# Autodesk Inventor assembly: side_channel
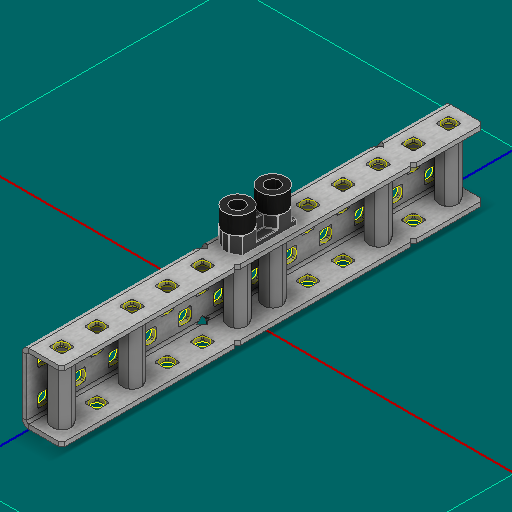
[picture p0: Inventor's stored thumbnail of the model, 512x512]
Saved by Autodesk Inventor 2025 (Build 290162000, 162)
## iProperties
Created: 2024-08-17
Part Number: side_channel
Document SubType Name: Assembly
Designer: averey
Author: averey
## Documents named in this file (9)
- C:\Users\avere\vex_robotics_high_stakes\hardware\cad\ATLAS\chassis\structure\side_channel.iam
- C:\Users\avere\vex_robotics_high_stakes\hardware\cad\VEX-CAD-Inventor\Structure\Standoff\Standoff .875.ipt
- C:\Users\avere\vex_robotics_high_stakes\hardware\cad\VEX-CAD-Inventor\Structure\Standoff.ipt
- C:\Users\avere\vex_robotics_high_stakes\hardware\cad\VEX-CAD-Inventor\Motion\Spacers\Spacer Nylon .375 OD.ipt
- C:\Users\avere\vex_robotics_high_stakes\hardware\cad\VEX-CAD-Inventor\Structure\Hardware\Screw Steel - Star\SScrew Star Smooth .290.ipt
- C:\Users\avere\vex_robotics_high_stakes\hardware\cad\VEX-CAD-Inventor\Structure\Hardware\Screw Steel - Star.ipt
- C:\Users\avere\vex_robotics_high_stakes\hardware\cad\VEX-CAD-Inventor\Motion\Spacers\Spacer Nylon .375 OD\NSpacer .375 OD x .250.ipt
- C:\Users\avere\vex_robotics_high_stakes\hardware\cad\custom_parts\modified_parts\Bearing Flat Low Profile 2-Hole.ipt
- C:\Users\avere\vex_robotics_high_stakes\hardware\cad\VEX-CAD-Inventor\Structure\C Channel\Aluminum 1x2x1\Alu C 1x2x1x12.ipt
## Components (12 placed, 5 different names)
1. Standoff .875:1 — Insert:15
2. Standoff .875:2 — Insert:14, Insert:16, Mate:1
3. SScrew Star Smooth .290:1 — Insert:15
4. SScrew Star Smooth .290:2 — Insert:16
5. NSpacer .375 OD x .250:1 — Insert:8
6. NSpacer .375 OD x .250:2 — Insert:9, Mate:1
7. Bearing Flat Low Profile 2-Hole:1 — Insert:8, Insert:9, Insert:17
8. Standoff .875:3 — Insert:11
9. Standoff .875:4 — Insert:10
10. Standoff .875:5 — Insert:12
11. Standoff .875:6 — Insert:13
12. Alu C 1x2x1x12:1 — Insert:10, Insert:11, Insert:12, Insert:13, Insert:14, Insert:17
## Relationships (11: Insert 10, Mate 1)
- Insert:8 (1.27 mm): NSpacer .375 OD x .250:1 ↔ Bearing Flat Low Profile 2-Hole:1
- Insert:9 (1.27 mm): NSpacer .375 OD x .250:2 ↔ Bearing Flat Low Profile 2-Hole:1
- Insert:10: Standoff .875:4 ↔ Alu C 1x2x1x12:1
- Insert:11: Standoff .875:3 ↔ Alu C 1x2x1x12:1
- Insert:12: Standoff .875:5 ↔ Alu C 1x2x1x12:1
- Insert:13: Standoff .875:6 ↔ Alu C 1x2x1x12:1
- Insert:14: Standoff .875:2 ↔ Alu C 1x2x1x12:1
- Insert:15 (1.5875 mm): Standoff .875:1 ↔ SScrew Star Smooth .290:1
- Insert:16 (1.5875 mm): Standoff .875:2 ↔ SScrew Star Smooth .290:2
- Insert:17: Bearing Flat Low Profile 2-Hole:1 ↔ Alu C 1x2x1x12:1
- Mate:1: Standoff .875:2 ↔ NSpacer .375 OD x .250:2
